# Autodesk Inventor assembly: VNA-Port2-Kabelfixierung
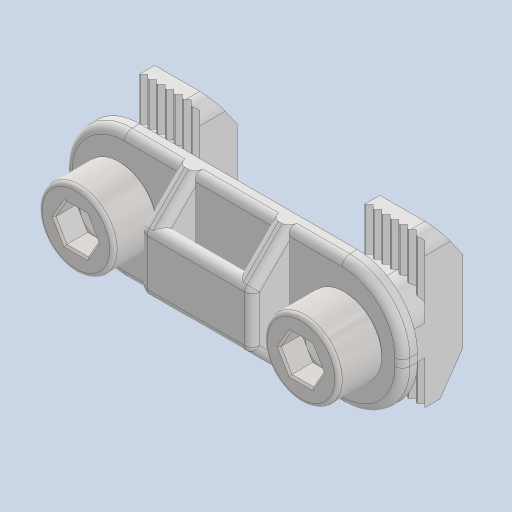
[picture p0: Inventor's stored thumbnail of the model, 512x512]
Saved by Autodesk Inventor 2023.2 (Build 272271000, 271)
## iProperties
Created: 2024-07-03
Part Number: VNA-Port2-Kabelfixierung
Document SubType Name: Assembly
Designer: Nils Bade
Author: Nils Bade
## Documents named in this file (4)
- C:\Users\nilsb\Documents\Inventor\Projektarbeit-Bade\RatRig_modified\VNA-Port2-Kabelfixierung.iam
- C:\Users\nilsb\Documents\Inventor\Projektarbeit-Bade\RatRig_modified\VNA-Port2-Kabelfixierung.ipt
- C:\Users\nilsb\Documents\Inventor\Projektarbeit-Bade\Schrauben\Cap Head Screw M6x12 v2.ipt
- C:\Users\nilsb\Documents\Inventor\Projektarbeit-Bade\RatRig_modified\T-NUT - DropIn 4040 SERIES - M6.ipt
## Components (5 placed, 3 different names)
1. VNA-Port2-Kabelfixierung:1 — Passend:1, Passend:2, Passend:3, Passend:4, Winkel:3, Winkel:4, Passend:11, Passend:12
2. Cap Head Screw M6x12 v2:1 — Passend:1, Passend:3, Passend:9
3. Cap Head Screw M6x12 v2:2 — Passend:2, Passend:4, Passend:10
4. T-NUT - DROP IN TYPE FOR 40 SERIES - M6:2 — Passend:10, Winkel:3, Passend:11
5. T-NUT - DROP IN TYPE FOR 40 SERIES - M6:1 — Passend:9, Winkel:4, Passend:12
## Relationships (16: Mate 12, Angle 4)
- Passend:1 [Mate]: VNA-Port2-Kabelfixierung:1 ↔ Cap Head Screw M6x12 v2:1
- Passend:2 [Mate]: VNA-Port2-Kabelfixierung:1 ↔ Cap Head Screw M6x12 v2:2
- Passend:3 [Mate]: VNA-Port2-Kabelfixierung:1 ↔ Cap Head Screw M6x12 v2:1
- Passend:4 [Mate]: VNA-Port2-Kabelfixierung:1 ↔ Cap Head Screw M6x12 v2:2
- [Mate]: Cap Head Screw M6x12 v2:2 ↔ T-NUT - DROP IN TYPE FOR 40 SERIES - M6:2
- [Mate]: Cap Head Screw M6x12 v2:1 ↔ T-NUT - DROP IN TYPE FOR 40 SERIES - M6:1
- [Angle] (0 deg): VNA-Port2-Kabelfixierung:1 ↔ T-NUT - DROP IN TYPE FOR 40 SERIES - M6:1
- [Angle] (0 deg): VNA-Port2-Kabelfixierung:1 ↔ T-NUT - DROP IN TYPE FOR 40 SERIES - M6:2
- [Mate] (4.5 mm): VNA-Port2-Kabelfixierung:1 ↔ T-NUT - DROP IN TYPE FOR 40 SERIES - M6:2
- [Mate] (4.5 mm): VNA-Port2-Kabelfixierung:1 ↔ T-NUT - DROP IN TYPE FOR 40 SERIES - M6:1
- Passend:9 [Mate]: Cap Head Screw M6x12 v2:1 ↔ T-NUT - DROP IN TYPE FOR 40 SERIES - M6:1
- Passend:10 [Mate]: Cap Head Screw M6x12 v2:2 ↔ T-NUT - DROP IN TYPE FOR 40 SERIES - M6:2
- Winkel:3 [Angle] (0 deg): VNA-Port2-Kabelfixierung:1 ↔ T-NUT - DROP IN TYPE FOR 40 SERIES - M6:2
- Winkel:4 [Angle] (0 deg): VNA-Port2-Kabelfixierung:1 ↔ T-NUT - DROP IN TYPE FOR 40 SERIES - M6:1
- Passend:11 [Mate] (4.5 mm): VNA-Port2-Kabelfixierung:1 ↔ T-NUT - DROP IN TYPE FOR 40 SERIES - M6:2
- Passend:12 [Mate] (4.5 mm): VNA-Port2-Kabelfixierung:1 ↔ T-NUT - DROP IN TYPE FOR 40 SERIES - M6:1
